# Autodesk Inventor assembly: Сальник
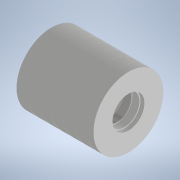
[picture p0: Inventor's stored thumbnail of the model, 180x180]
Saved by Autodesk Inventor 2021 (Build 250183000, 183)
## iProperties
Created: 2020-12-05
Part Number: Сальник
Document SubType Name: Assembly
Designer: Тимоха
Author: Тимоха
## Documents named in this file (7)
- C:\Users\Тимоха\Desktop\КР Компрессор\compressor\Сальник.iam
- C:\Users\Тимоха\Desktop\КР Компрессор\compressor\Дроссельное кольцо.ipt
- C:\Users\Тимоха\Desktop\КР Компрессор\compressor\Корпус дросселя.ipt
- C:\Users\Тимоха\Desktop\КР Компрессор\compressor\Пружина дросселя.ipt
- C:\Users\Тимоха\Desktop\КР Компрессор\compressor\Кольцо сальника.ipt
- C:\Users\Тимоха\Desktop\КР Компрессор\compressor\Корпус сальника.ipt
- C:\Users\Тимоха\Desktop\КР Компрессор\compressor\Пружина сальника.ipt
## Components (45 placed, 6 different names)
1. Дроссельное кольцо:1
2. Корпус дросселя:1
3. Пружина дросселя:1
4. Кольцо сальника:1
5. Корпус сальника:1
6. Пружина сальника:1
7. Кольцо сальника:2
8. Пружина сальника:2
9. Кольцо сальника:3
10. Пружина сальника:3
11. Кольцо сальника:4
12. Корпус сальника:2
13. Пружина сальника:4
14. Кольцо сальника:5
15. Пружина сальника:5
16. Кольцо сальника:6
17. Пружина сальника:6
18. Кольцо сальника:7
19. Корпус сальника:3
20. Пружина сальника:7
21. Кольцо сальника:8
22. Пружина сальника:8
23. Кольцо сальника:9
24. Пружина сальника:9
25. Кольцо сальника:10
26. Корпус сальника:4
27. Пружина сальника:10
28. Кольцо сальника:11
29. Пружина сальника:11
30. Кольцо сальника:12
31. Пружина сальника:12
32. Кольцо сальника:13
33. Корпус сальника:5
34. Пружина сальника:13
35. Кольцо сальника:14
36. Пружина сальника:14
37. Кольцо сальника:15
38. Пружина сальника:15
39. Кольцо сальника:16
40. Корпус сальника:6
41. Пружина сальника:16
42. Кольцо сальника:17
43. Пружина сальника:17
44. Кольцо сальника:18
45. Пружина сальника:18
## Relationships (42: WeldJoint 42)
- [WeldJoint] (2 mm): Дроссельное кольцо:1 ↔ Пружина дросселя:1
- [WeldJoint]: Дроссельное кольцо:1 ↔ Корпус дросселя:1
- [WeldJoint] (-1 mm): Кольцо сальника:1 ↔ Пружина сальника:1
- [WeldJoint] (-1 mm): Кольцо сальника:2 ↔ Пружина сальника:2
- [WeldJoint] (-1 mm): Кольцо сальника:3 ↔ Пружина сальника:3
- [WeldJoint]: Кольцо сальника:2 ↔ Кольцо сальника:3
- [WeldJoint]: Кольцо сальника:1 ↔ Кольцо сальника:2
- [WeldJoint]: Корпус сальника:1 ↔ Кольцо сальника:3
- [WeldJoint] (-1 mm): Кольцо сальника:4 ↔ Пружина сальника:4
- [WeldJoint] (-1 mm): Кольцо сальника:5 ↔ Пружина сальника:5
- [WeldJoint] (-1 mm): Кольцо сальника:6 ↔ Пружина сальника:6
- [WeldJoint]: Кольцо сальника:5 ↔ Кольцо сальника:6
- [WeldJoint]: Кольцо сальника:4 ↔ Кольцо сальника:5
- [WeldJoint]: Корпус сальника:2 ↔ Кольцо сальника:6
- [WeldJoint] (-1 mm): Кольцо сальника:7 ↔ Пружина сальника:7
- [WeldJoint] (-1 mm): Кольцо сальника:8 ↔ Пружина сальника:8
- [WeldJoint] (-1 mm): Кольцо сальника:9 ↔ Пружина сальника:9
- [WeldJoint]: Кольцо сальника:8 ↔ Кольцо сальника:9
- [WeldJoint]: Кольцо сальника:7 ↔ Кольцо сальника:8
- [WeldJoint]: Корпус сальника:3 ↔ Кольцо сальника:9
- [WeldJoint] (-1 mm): Кольцо сальника:10 ↔ Пружина сальника:10
- [WeldJoint] (-1 mm): Кольцо сальника:11 ↔ Пружина сальника:11
- [WeldJoint] (-1 mm): Кольцо сальника:12 ↔ Пружина сальника:12
- [WeldJoint]: Кольцо сальника:11 ↔ Кольцо сальника:12
- [WeldJoint]: Кольцо сальника:10 ↔ Кольцо сальника:11
- [WeldJoint]: Корпус сальника:4 ↔ Кольцо сальника:12
- [WeldJoint] (-1 mm): Кольцо сальника:13 ↔ Пружина сальника:13
- [WeldJoint] (-1 mm): Кольцо сальника:14 ↔ Пружина сальника:14
- [WeldJoint] (-1 mm): Кольцо сальника:15 ↔ Пружина сальника:15
- [WeldJoint]: Кольцо сальника:14 ↔ Кольцо сальника:15
- [WeldJoint]: Кольцо сальника:13 ↔ Кольцо сальника:14
- [WeldJoint]: Корпус сальника:5 ↔ Кольцо сальника:15
- [WeldJoint] (-1 mm): Кольцо сальника:16 ↔ Пружина сальника:16
- [WeldJoint] (-1 mm): Кольцо сальника:17 ↔ Пружина сальника:17
- [WeldJoint] (-1 mm): Кольцо сальника:18 ↔ Пружина сальника:18
- [WeldJoint]: Кольцо сальника:17 ↔ Кольцо сальника:18
- [WeldJoint]: Кольцо сальника:16 ↔ Кольцо сальника:17
- [WeldJoint]: Корпус сальника:6 ↔ Кольцо сальника:18
- [WeldJoint]: Корпус сальника:1 ↔ Корпус сальника:6
- [WeldJoint]: Корпус сальника:3 ↔ Корпус сальника:6
- [WeldJoint]: Корпус сальника:4 ↔ Корпус сальника:5
- [WeldJoint]: Корпус сальника:2 ↔ Корпус сальника:5
## Named parameters: d81_d45_d35 = -1 mm, d82_d46_d36_d35 = -1 mm, d83_d47_d37_d35 = -1 mm, d84_d48_d38 = 0 mm, d85_d49_d39 = 0 mm, d86_d50_d40 = 0 mm, d53_d45_d35 = -1 mm, d54_d46_d36_d35 = -1 mm, d55_d47_d37_d35 = -1 mm, d56_d48_d38 = 0 mm, d57_d49_d39 = 0 mm, d58_d50_d40 = 0 mm, d60_d45_d35 = -1 mm, d61_d46_d36_d35 = -1 mm, d62_d47_d37_d35 = -1 mm, d63_d48_d38 = 0 mm, d64_d49_d39 = 0 mm, d65_d50_d40 = 0 mm, d67_d45_d35 = -1 mm, d68_d46_d36_d35 = -1 mm, d69_d47_d37_d35 = -1 mm, d70_d48_d38 = 0 mm, d71_d49_d39 = 0 mm, d72_d50_d40 = 0 mm, d74_d45_d35 = -1 mm, d75_d46_d36_d35 = -1 mm, d76_d47_d37_d35 = -1 mm, d77_d48_d38 = 0 mm, d78_d49_d39 = 0 mm, d79_d50_d40 = 0 mm, d34_d41 = 2 mm, d45_d35 = -1 mm, d46_d36_d35 = -1 mm, d47_d37_d35 = -1 mm, d48_d38 = 0 mm, d49_d39 = 0 mm, d50_d40 = 0 mm
